# Autodesk Inventor assembly: Assembly2
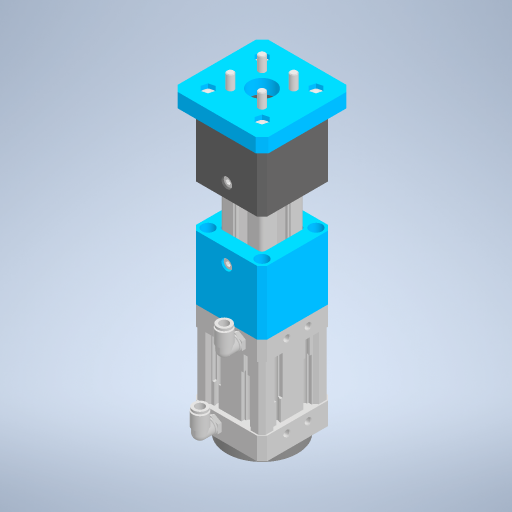
[picture p0: Inventor's stored thumbnail of the model, 512x512]
Saved by Autodesk Inventor 2023 (Build 270158000, 158)
## iProperties
Created: 2022-05-24
Part Number: Assembly2
Document SubType Name: Assembly
Designer: romanp
Author: romanp
## Documents named in this file (12)
- C:\Users\romanp\Downloads\SMC_EE_MHM-32D1-X6400\Pack_and_Go\Assembly_SMC_EE.iam
- C:\Users\romanp\Downloads\SMC_EE_MHM-32D1-X6400\Pack_and_Go\MHM-32D1-X6400(0).iam
- C:\Users\romanp\Downloads\SMC_EE_MHM-32D1-X6400\Pack_and_Go\Part_Top_a_Blue.ipt
- C:\Users\romanp\Downloads\SMC_EE_MHM-32D1-X6400\Pack_and_Go\Part_Bottom_Blue.ipt
- C:\Users\romanp\Downloads\SMC_EE_MHM-32D1-X6400\Pack_and_Go\Part_Middle_Black.ipt
- C:\Users\romanp\Downloads\SMC_EE_MHM-32D1-X6400\Pack_and_Go\ITEM30x30x100.ipt
- C:\Users\romanp\Downloads\SMC_EE_MHM-32D1-X6400\Pack_and_Go\M5x25.ipt
- C:\Users\romanp\Downloads\SMC_EE_MHM-32D1-X6400\Pack_and_Go\M4_nut.ipt
- C:\Users\romanp\Downloads\SMC_EE_MHM-32D1-X6400\Pack_and_Go\M4x10.ipt
- C:\Users\romanp\Downloads\SMC_EE_MHM-32D1-X6400\Pack_and_Go\M5x20.ipt
- C:\Users\romanp\Downloads\SMC_EE_MHM-32D1-X6400\Pack_and_Go\M4x20.ipt
- C:\Users\romanp\Downloads\SMC_EE_MHM-32D1-X6400\Pack_and_Go\KQ2L06-01N.ipt
## Components (27 placed, 12 different names)
1. Part_Top_a_Blue — Insert:25, Insert:45, Insert:46, Insert:47, Insert:54
2. M5x25:1
3. M4x10:5
4. M4x20:1
5. M4_nut:3 — Insert:25
6. M4x10:7
7. ITEM30x30x100:3
8. MHM-32D1-X6400(0):3 [sub-assembly] — Insert:51, Insert:52, Insert:53
9. M5x75:2
10. M4x10:8
11. M4x10:9
12. M5x75:3
13. M5x75:4
14. M5x75:5
15. M5x25:2
16. M5x25:3
17. M5x25:4
18. M4_nut:4 — Insert:46
19. M4_nu:5 — Insert:47
20. M4_nu:6 — Insert:45
21. M4x20:5
22. M4x20:6
23. M4x20:7
24. KQ2L06-01N:3 — Insert:51
25. KQ2L06-01N:4 — Insert:52
26. Part_Middle_Black:1 — Insert:54
27. Part_Bottom_Blue:1 — Insert:53
## Relationships (8: Insert 8)
- Insert:25: Part_Top_a_Blue ↔ M4_nut:3
- Insert:45: Part_Top_a_Blue ↔ M4_nu:6
- Insert:46: Part_Top_a_Blue ↔ M4_nut:4
- Insert:47: Part_Top_a_Blue ↔ M4_nu:5
- Insert:51: MHM-32D1-X6400(0):3 ↔ KQ2L06-01N:3
- Insert:52: MHM-32D1-X6400(0):3 ↔ KQ2L06-01N:4
- Insert:53: MHM-32D1-X6400(0):3 ↔ Part_Bottom_Blue:1
- Insert:54: Part_Top_a_Blue ↔ Part_Middle_Black:1
